# Autodesk Inventor assembly: CuboidSecurityBoxOpenedLayer
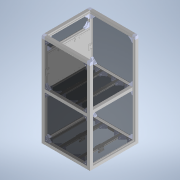
[picture p0: Inventor's stored thumbnail of the model, 180x180]
Saved by Autodesk Inventor 2021 (Build 250183000, 183)
## iProperties
Created: 2020-11-09
Part Number: CuboidSecurityBoxOpenedLayer
Document SubType Name: Assembly
Designer: gisen
Author: gisen
## Documents named in this file (3)
- D:\GitProjects\CAD-Data\CuboidAccessories\SecurityBox\CuboidSecurityBoxOpenedLayer.iam
- D:\GitProjects\CAD-Data\CuboidAccessories\SecurityBox\Assemblies\CuboidSecurityBoxBasis.iam
- D:\GitProjects\CAD-Data\CuboidAccessories\SecurityBox\Assemblies\AdditionalLayerAssembly.iam
## Components (2 placed, 2 different names)
1. CuboidSecurityBoxBasis:1 [sub-assembly] — フラッシュ:1, メイト:1, フラッシュ:2, フラッシュ:3, フラッシュ:4, フラッシュ:5
2. AdditionalLayerAssembly:1 [sub-assembly] — フラッシュ:1, メイト:1, フラッシュ:2
## Relationships (6: Flush 5, Mate 1)
- フラッシュ:1 [Flush] (20 mm): CuboidSecurityBoxBasis:1 ↔ AdditionalLayerAssembly:1
- メイト:1 [Mate]: CuboidSecurityBoxBasis:1 ↔ AdditionalLayerAssembly:1
- フラッシュ:2 [Flush]: CuboidSecurityBoxBasis:1 ↔ AdditionalLayerAssembly:1
- フラッシュ:3 [Flush]: CuboidSecurityBoxBasis:1
- フラッシュ:4 [Flush]: CuboidSecurityBoxBasis:1
- フラッシュ:5 [Flush]: CuboidSecurityBoxBasis:1
